# Autodesk Inventor assembly: batprotect_assembly
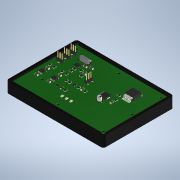
[picture p0: Inventor's stored thumbnail of the model, 180x180]
Saved by Autodesk Inventor 2021.3 (Build 253353000, 353)
## iProperties
Created: 2022-01-18
Part Number: batprotect_assembly
Document SubType Name: Assembly
Designer: nxf77172
Author: nxf77172
## Documents named in this file (3)
- C:\Users\nxf77172\OneDrive - NXP\ROSinante\Mechanical\batprotect_assembly.iam
- C:\Users\nxf77172\NXP\Sabine Kokot - ender5pro\Ender+5+X+Carriage\files\BProtect-Case-Body.ipt
- C:\Users\nxf77172\OneDrive - NXP\ROSinante\Electrical\Battery-protector\Battery-protector.iam
## Components (2 placed, 2 different names)
1. BProtect-Case-Body:1 — Mate:1, Mate:2
2. Battery-protector:1 [sub-assembly] — Mate:1, Mate:2
## Relationships (2: Mate 2)
- Mate:1: BProtect-Case-Body:1 ↔ Battery-protector:1
- Mate:2: BProtect-Case-Body:1 ↔ Battery-protector:1
